# Autodesk Inventor assembly: Assembly1
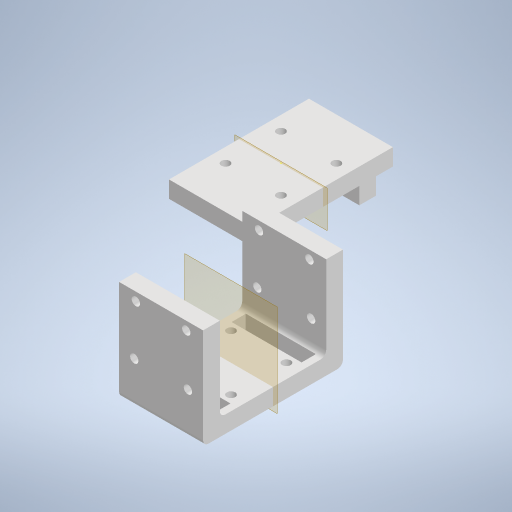
[picture p0: Inventor's stored thumbnail of the model, 512x512]
Saved by Autodesk Inventor 2023 (Build 270158000, 158)
## iProperties
Created: 2022-04-22
Part Number: Assembly1
Document SubType Name: Assembly
Designer: Maarten
Author: Maarten
## Documents named in this file (3)
- C:\Users\Maarten\Documents\IIW\3ba\BachProef\3D\Assembly1.iam
- C:\Users\Maarten\Documents\IIW\3ba\BachProef\3D\MGN_Plate.ipt
- C:\Users\Maarten\Documents\IIW\3ba\BachProef\3D\PanelHolder.ipt
## Components (2 placed, 2 different names)
1. MGN_Plate:1 — Mate:1, Mate:2, Mate:3
2. PanelHolder:1 — Mate:1, Mate:2, Mate:3
## Relationships (3: Mate 3)
- Mate:1: MGN_Plate:1 ↔ PanelHolder:1
- Mate:2: MGN_Plate:1 ↔ PanelHolder:1
- Mate:3: MGN_Plate:1 ↔ PanelHolder:1
